# Autodesk Inventor assembly: Modbay
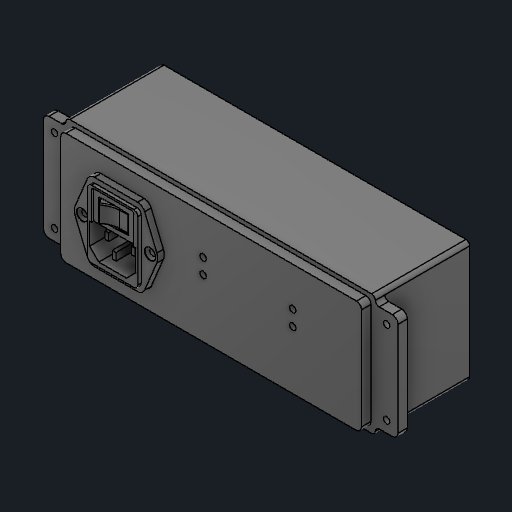
[picture p0: Inventor's stored thumbnail of the model, 512x512]
Saved by Autodesk Inventor 2026.2 (Build 302298000, 298)
## iProperties
Created: 2026-08-18
Part Number: Modbay
Document SubType Name: Assembly
Designer: JoshuaEah
Author: JoshuaEah
## Documents named in this file (4)
- C:\Users\JoshuaEah\Documents\GitHub\Designed-Trinkets\Guitar\Modular Pedalboard\Modbay.iam
- C:\Users\JoshuaEah\Documents\GitHub\Designed-Trinkets\Guitar\Modular Pedalboard\Junction Box Modbay.ipt
- C:\Users\JoshuaEah\Documents\GitHub\Designed-Trinkets\Guitar\Modular Pedalboard\Hardware\C14 Inlet.ipt
- C:\Users\JoshuaEah\Documents\GitHub\Designed-Trinkets\Guitar\Modular Pedalboard\Hardware\Terminal Block.ipt
## Components (3 placed, 3 different names)
1. Junction Box Modbay:1 — Insert:1, Insert:2, Insert:3
2. C14 Inlet:1 — Insert:1
3. Terminal Block:1 — Insert:2, Insert:3
## Relationships (3: Insert 3)
- Insert:1: Junction Box Modbay:1 ↔ C14 Inlet:1
- Insert:2: Junction Box Modbay:1 ↔ Terminal Block:1
- Insert:3: Junction Box Modbay:1 ↔ Terminal Block:1
